# Autodesk Inventor assembly: under_body
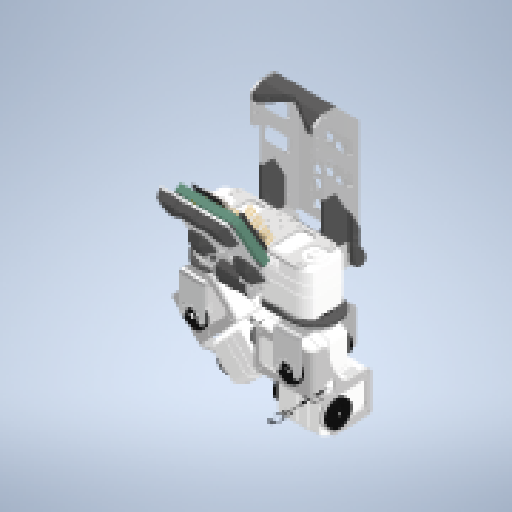
[picture p0: Inventor's stored thumbnail of the model, 512x512]
Saved by Autodesk Inventor 2024.1 (Build 281209000, 209)
## iProperties
Created: 2024-10-10
Part Number: under_body
Document SubType Name: Assembly
Designer: hibik
Author: hibik
## Documents named in this file (9)
- C:\Users\hibik\Documents\Robomech\HR\Eglantyne\hard\under_body\under_body.iam
- C:\Users\hibik\Documents\Robomech\HR\Eglantyne\hard\under_body\hipjoint.iam
- C:\Users\hibik\Documents\Robomech\HR\Eglantyne\hard\under_body\yaw_joint.ipt
- C:\Users\hibik\Documents\Robomech\HR\Eglantyne\hard\under_body\to_leg\hipjoint_toleg_right.iam
- C:\Users\hibik\Documents\Robomech\HR\Eglantyne\hard\common_parts\joint_setter_c.ipt
- C:\Users\hibik\Documents\Robomech\HR\Eglantyne\hard\common_parts\joint_setter_s.ipt
- C:\Users\hibik\Documents\Robomech\HR\Eglantyne\hard\under_body\to_leg\hipjoint_toleg_left.iam
- C:\Users\hibik\Documents\Robomech\HR\Eglantyne\hard\under_body\board_setter\board_setter.iam
- C:\Users\hibik\Documents\Robomech\HR\Eglantyne\hard\under_body\battery_cover\battery_cover.iam
## Components (11 placed, 8 different names)
1. hipjoint:1 [sub-assembly] — 挿入:7, 挿入:13, 挿入:15, 角度:1, 挿入:16, メイト:1
2. yaw_joint:1 — 挿入:2, 挿入:3, 挿入:4
3. hipjoint_toleg_right:1 [sub-assembly] — 挿入:2
4. joint_setter_c:1 — 挿入:5, 挿入:6
5. joint_setter_s:1 — 挿入:3, 挿入:4, 挿入:5, 挿入:6, 挿入:7
6. yaw_joint:2 — 挿入:14
7. joint_setter_c:2 — 挿入:12
8. joint_setter_s:2 — 挿入:12, 挿入:13
9. hipjoint_toleg_left:1 [sub-assembly] — 挿入:14
10. board_setter:1 [sub-assembly] — 挿入:15, 角度:1
11. battery_cover:1 [sub-assembly] — 挿入:16, メイト:1
## Relationships (17: Insert 15, Angle 1, Mate 1)
- 挿入:2 [Insert]: yaw_joint:1 ↔ hipjoint_toleg_right:1
- 挿入:3 [Insert]: yaw_joint:1 ↔ joint_setter_s:1
- 挿入:4 [Insert]: yaw_joint:1 ↔ joint_setter_s:1
- 挿入:5 [Insert]: joint_setter_c:1 ↔ joint_setter_s:1
- 挿入:6 [Insert]: joint_setter_c:1 ↔ joint_setter_s:1
- 挿入:7 [Insert]: hipjoint:1 ↔ joint_setter_s:1
- [Insert]: yaw_joint:2 ↔ joint_setter_s:2
- [Insert]: yaw_joint:2 ↔ joint_setter_s:2
- [Insert]: joint_setter_c:2 ↔ joint_setter_s:2
- [Insert]: joint_setter_c:2 ↔ joint_setter_s:2
- 挿入:12 [Insert]: joint_setter_c:2 ↔ joint_setter_s:2
- 挿入:13 [Insert]: hipjoint:1 ↔ joint_setter_s:2
- 挿入:14 [Insert]: yaw_joint:2 ↔ hipjoint_toleg_left:1
- 挿入:15 [Insert] (0.5 mm): hipjoint:1 ↔ board_setter:1
- 角度:1 [Angle] (0 deg): hipjoint:1 ↔ board_setter:1
- 挿入:16 [Insert] (0.5 mm): hipjoint:1 ↔ battery_cover:1
- メイト:1 [Mate]: hipjoint:1 ↔ battery_cover:1
## Named parameters: d7_d2 = 0 mm, d8_d3 = 0 mm, d9_d4 = 0 mm, d10_d5 = 0 mm
